# Autodesk Inventor assembly: Robot
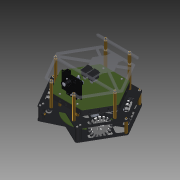
[picture p0: Inventor's stored thumbnail of the model, 180x180]
Saved by Autodesk Inventor 2015 (Build 190159000, 159)
## iProperties
Created: 2016-10-01
Part Number: Robot
Document SubType Name: Assembly
Designer: James Yelland
Author: James Yelland
## Documents named in this file (26)
- C:\Users\James Yelland\git\LJ-STAND\Design\Models\Robot\Robot.iam
- C:\Users\James Yelland\git\LJ-STAND\Design\Models\Robot\Bottom Plate.ipt
- C:\Users\James Yelland\git\LJ-STAND\Design\Models\Robot\Motor Mount.ipt
- C:\Users\James Yelland\git\LJ-STAND\Design\Models\Fasteners\Standoff 30 M-F.ipt
- C:\Users\James Yelland\git\LJ-STAND\Design\Models\Robot\LDR mount.ipt
- C:\Users\James Yelland\git\LJ-STAND\Design\Models\Robot\Laser diode mount.ipt
- C:\Users\James Yelland\git\LJ-STAND\Design\Models\Fasteners\M3x10 Screw.ipt
- C:\Users\James Yelland\git\LJ-STAND\Design\Models\Robot\Motor Support.ipt
- C:\Users\James Yelland\git\LJ-STAND\Design\Models\Fasteners\M3 Hex Nut.ipt
- C:\Users\James Yelland\git\LJ-STAND\Design\Models\Common\Imported Components\maxon_PN_0_1\maxon_PN_0_1.iam
- C:\Users\James Yelland\git\LJ-STAND\Design\Models\Fasteners\M2x4 Screw.ipt
- C:\Users\James Yelland\git\LJ-STAND\Design\Models\Robot\Light Sensor PCB.ipt
- C:\Users\James Yelland\git\LJ-STAND\Design\Models\Common\Wheel.ipt
- C:\Users\James Yelland\git\LJ-STAND\Design\Models\Robot\Middle Plate.ipt
- C:\Users\James Yelland\git\LJ-STAND\Design\Models\Fasteners\Standoff 10 M-F.ipt
- C:\Users\James Yelland\git\LJ-STAND\Design\Models\Robot\TSOP Cover Ring.ipt
- C:\Users\James Yelland\git\LJ-STAND\Design\Models\Robot\Main PCB.ipt
- C:\Users\James Yelland\git\LJ-STAND\Design\Models\Fasteners\M3x20 Screw.ipt
- C:\Users\James Yelland\git\LJ-STAND\Design\Models\Fasteners\Standoff 50 M-F.ipt
- C:\Users\James Yelland\git\LJ-STAND\Design\Models\Robot\Top Plate.ipt
- C:\Users\James Yelland\git\LJ-STAND\Design\Models\Fasteners\Standoff 20 M-F.ipt
- C:\Users\James Yelland\git\LJ-STAND\Design\Models\Robot\Handle.ipt
- C:\Users\James Yelland\git\LJ-STAND\Design\Models\Common\Laser Diode.ipt
- C:\Users\James Yelland\git\LJ-STAND\Design\Models\Common\Pixy angle bracket.ipt
- C:\Users\James Yelland\git\LJ-STAND\Design\Models\Pixy\pixy\Imported Components\Pixy(CMUcam5)\Pixy(CMUcam5).iam
- C:\Users\James Yelland\git\LJ-STAND\Design\Models\Common\Toggle switch.ipt
## Components (102 placed, 25 different names)
1. Bottom Plate:1 — Insert:1, Insert:2, Insert:3, Insert:4, Insert:5, Insert:6, Insert:7, Insert:8, Mate:1, Mate:2, Mate:3, Mate:4, Mate:5, Mate:6, Mate:7, Mate:8, Mate:9, Mate:10, Mate:11, Mate:12, Insert:9, Insert:10, Insert:11, Insert:12, Insert:31, Insert:32, Insert:33, Insert:34, Insert:35, Insert:36, Insert:37, Insert:38, Insert:39, Insert:40, Insert:45, Insert:46, Insert:47, Insert:48
2. Motor Mount:1 — Mate:2, Mate:7, Mate:8, Insert:15, Mate:13, Insert:25, Insert:26, Insert:27
3. Motor Mount:2 — Mate:1, Mate:5, Mate:6, Insert:16, Mate:14, Insert:22, Insert:23, Insert:24
4. Motor Mount:3 — Mate:3, Mate:9, Mate:10, Insert:18, Mate:15, Insert:19, Insert:20, Insert:21
5. Motor Mount:4 — Mate:4, Mate:11, Mate:12, Insert:17, Mate:16, Insert:28, Insert:29, Insert:30
6. Standoff 30 M-F:1 — Insert:3
7. Standoff 30 M-F:2 — Insert:4
8. Standoff 30 M-F:3 — Insert:2, Insert:50
9. Standoff 30 M-F:4 — Insert:1, Insert:49
10. LDR mount:1 — Insert:33, Insert:34
11. Laser diode mount:1 — Insert:31, Insert:32, Insert:93
12. M3x10 Screw:1 — Insert:5
13. M3x10 Screw:2 — Insert:7
14. M3x10 Screw:3 — Insert:6
15. M3x10 Screw:4 — Insert:8
16. Motor Support:1 — Insert:9, Insert:10, Insert:13, Insert:14
17. M3 Hex Nut:1 — Insert:13
18. M3x10 Screw:5 — Insert:12
19. M3 Hex Nut:2 — Insert:14
20. M3x10 Screw:6 — Insert:11
21. maxon_PN_0_1:1 [sub-assembly] — Insert:16, Mate:14, Mate:18, Flush:2
22. maxon_PN_0_1:2 [sub-assembly] — Insert:17, Mate:16, Mate:20, Flush:4
23. maxon_PN_0_1:3 [sub-assembly] — Insert:15, Mate:13, Mate:19, Flush:3
24. maxon_PN_0_1:4 [sub-assembly] — Insert:18, Mate:15, Mate:17, Flush:1
25. M2x4 Screw:1 — Insert:25
26. M2x4 Screw:3 — Insert:19
27. M2x4 Screw:4 — Insert:28
28. M2x4 Screw:5 — Insert:27
29. M2x4 Screw:6 — Insert:26
30. M2x4 Screw:7 — Insert:24
31. M2x4 Screw:8 — Insert:21
32. M2x4 Screw:9 — Insert:20
33. M2x4 Screw:10 — Insert:29
34. M2x4 Screw:11 — Insert:23
35. M2x4 Screw:12 — Insert:22
36. M2x4 Screw:13 — Insert:30
37. Light Sensor PCB:1 — Insert:35, Insert:36, Insert:41, Insert:42, Insert:43, Insert:44
38. M3 Hex Nut:3 — Insert:41
39. M3x10 Screw:7 — Insert:37
40. M3 Hex Nut:4 — Insert:42
41. M3x10 Screw:8 — Insert:38
42. M3 Hex Nut:5 — Insert:43
43. M3x10 Screw:9 — Insert:39
44. M3 Hex Nut:6 — Insert:44
45. M3x10 Screw:10 — Insert:40
46. M3x10 Screw:11 — Insert:45
47. M3x10 Screw:12 — Insert:46
48. M3x10 Screw:13 — Insert:47
49. M3x10 Screw:14 — Insert:48
50. Wheel:1 — Mate:18, Flush:2
51. Wheel:2 — Mate:19, Flush:3
52. Wheel:3 — Mate:17, Flush:1
53. Wheel:4 — Mate:20, Flush:4
54. Middle Plate:1 — Insert:49, Insert:50, Insert:51, Insert:52, Insert:53, Insert:54, Insert:55, Insert:56, Insert:57, Insert:58, Insert:59, Insert:60, Insert:61, Insert:62, Insert:63, Insert:64, Insert:65, Insert:66, Insert:75, Insert:76, Insert:77, Insert:78, Insert:79, Insert:80, Insert:81, Insert:82, Insert:98, Insert:99
55. M3 Hex Nut:7 — Insert:55
56. M3x10 Screw:15 — Insert:51
57. M3 Hex Nut:8 — Insert:56
58. M3x10 Screw:16 — Insert:52
59. M3 Hex Nut:9 — Insert:57
60. M3x10 Screw:17 — Insert:53
61. M3 Hex Nut:10 — Insert:58
62. M3x10 Screw:18 — Insert:54
63. Standoff 10 M-F:1 — Insert:59
64. Standoff 10 M-F:2 — Insert:60
65. Standoff 10 M-F:3 — Insert:61, Insert:67
66. Standoff 10 M-F:4 — Insert:62, Insert:68
67. M3 Hex Nut:11 — Insert:65
68. M3 Hex Nut:12 — Insert:66
69. M3 Hex Nut:13 — Insert:64
70. M3 Hex Nut:14 — Insert:63
71. TSOP Cover Ring:1 — Insert:67, Insert:68, Insert:69, Insert:70
72. Main PCB:1 — Insert:69, Insert:70, Insert:71, Insert:72, Insert:73, Insert:74, Insert:94, Insert:95
73. M3x20 Screw:1 — Insert:74
74. M3x20 Screw:2 — Insert:73
75. M3x20 Screw:3 — Insert:72
76. M3x20 Screw:4 — Insert:71
77. M3x10 Screw:19 — Insert:82
78. Standoff 50 M-F:1 — Insert:75, Insert:83
79. M3x10 Screw:20 — Insert:81
80. Standoff 50 M-F:2 — Insert:76, Insert:84
81. M3x10 Screw:21 — Insert:80
82. Standoff 50 M-F:3 — Insert:77
83. M3x10 Screw:22 — Insert:79
84. Standoff 50 M-F:4 — Insert:78
85. Top Plate:1 — Insert:83, Insert:84, Insert:85, Insert:86, Insert:91, Insert:92, Mate:21, Mate:22, Mate:23, Mate:24, Mate:25, Mate:26, Insert:100, Insert:101
86. Standoff 20 M-F:1 — Insert:85, Insert:87
87. Standoff 20 M-F:2 — Insert:86, Insert:88
88. Handle:1 — Insert:87, Insert:88, Insert:89, Insert:90
89. M3 Hex Nut:15 — Insert:89
90. M3 Hex Nut:16 — Insert:90
91. M3 Hex Nut:17 — Insert:91
92. M3 Hex Nut:18 — Insert:92
93. Laser Diode:1 — Insert:93
94. Pixy angle bracket:1 — Insert:95, Insert:96
95. Pixy angle bracket:2 — Insert:94, Insert:97
96. Pixy(CMUcam5):1 [sub-assembly] — Insert:96, Insert:97
97. Toggle switch:1 — Mate:21, Mate:25, Mate:26
98. Toggle switch:2 — Mate:22, Mate:23, Mate:24
99. Standoff 50 M-F:5 — Insert:98
100. Standoff 50 M-F:6 — Insert:99
101. M3 Hex Nut:19 — Insert:100
102. M3 Hex Nut:20 — Insert:101
## Relationships (131: Insert 101, Mate 26, Flush 4)
- Insert:1: Bottom Plate:1 ↔ Standoff 30 M-F:4
- Insert:2: Bottom Plate:1 ↔ Standoff 30 M-F:3
- Insert:3: Bottom Plate:1 ↔ Standoff 30 M-F:1
- Insert:4: Bottom Plate:1 ↔ Standoff 30 M-F:2
- Insert:5: Bottom Plate:1 ↔ M3x10 Screw:1
- Insert:6: Bottom Plate:1 ↔ M3x10 Screw:3
- Insert:7: Bottom Plate:1 ↔ M3x10 Screw:2
- Insert:8: Bottom Plate:1 ↔ M3x10 Screw:4
- Mate:1: Bottom Plate:1 ↔ Motor Mount:2
- Mate:2: Bottom Plate:1 ↔ Motor Mount:1
- Mate:3: Bottom Plate:1 ↔ Motor Mount:3
- Mate:4: Bottom Plate:1 ↔ Motor Mount:4
- Mate:5: Bottom Plate:1 ↔ Motor Mount:2
- Mate:6: Bottom Plate:1 ↔ Motor Mount:2
- Mate:7: Bottom Plate:1 ↔ Motor Mount:1
- Mate:8: Bottom Plate:1 ↔ Motor Mount:1
- Mate:9: Bottom Plate:1 ↔ Motor Mount:3
- Mate:10: Bottom Plate:1 ↔ Motor Mount:3
- Mate:11: Bottom Plate:1 ↔ Motor Mount:4
- Mate:12: Bottom Plate:1 ↔ Motor Mount:4
- Insert:9: Bottom Plate:1 ↔ Motor Support:1
- Insert:10: Bottom Plate:1 ↔ Motor Support:1
- Insert:11: Bottom Plate:1 ↔ M3x10 Screw:6
- Insert:12: Bottom Plate:1 ↔ M3x10 Screw:5
- Insert:13: Motor Support:1 ↔ M3 Hex Nut:1
- Insert:14: Motor Support:1 ↔ M3 Hex Nut:2
- Insert:15: Motor Mount:1 ↔ maxon_PN_0_1:3
- Insert:16: Motor Mount:2 ↔ maxon_PN_0_1:1
- Insert:17: Motor Mount:4 ↔ maxon_PN_0_1:2
- Insert:18: Motor Mount:3 ↔ maxon_PN_0_1:4
- Mate:13: Motor Mount:1 ↔ maxon_PN_0_1:3
- Mate:14: Motor Mount:2 ↔ maxon_PN_0_1:1
- Mate:15: Motor Mount:3 ↔ maxon_PN_0_1:4
- Mate:16: Motor Mount:4 ↔ maxon_PN_0_1:2
- Insert:19: Motor Mount:3 ↔ M2x4 Screw:3
- Insert:20: Motor Mount:3 ↔ M2x4 Screw:9
- Insert:21: Motor Mount:3 ↔ M2x4 Screw:8
- Insert:22: Motor Mount:2 ↔ M2x4 Screw:12
- Insert:23: Motor Mount:2 ↔ M2x4 Screw:11
- Insert:24: Motor Mount:2 ↔ M2x4 Screw:7
- Insert:25: Motor Mount:1 ↔ M2x4 Screw:1
- Insert:26: Motor Mount:1 ↔ M2x4 Screw:6
- Insert:27: Motor Mount:1 ↔ M2x4 Screw:5
- Insert:28: Motor Mount:4 ↔ M2x4 Screw:4
- Insert:29: Motor Mount:4 ↔ M2x4 Screw:10
- Insert:30: Motor Mount:4 ↔ M2x4 Screw:13
- Insert:31: Bottom Plate:1 ↔ Laser diode mount:1
- Insert:32: Bottom Plate:1 ↔ Laser diode mount:1
- Insert:33: Bottom Plate:1 ↔ LDR mount:1
- Insert:34: Bottom Plate:1 ↔ LDR mount:1
- Insert:35: Bottom Plate:1 ↔ Light Sensor PCB:1
- Insert:36: Bottom Plate:1 ↔ Light Sensor PCB:1
- Insert:37: Bottom Plate:1 ↔ M3x10 Screw:7
- Insert:38: Bottom Plate:1 ↔ M3x10 Screw:8
- Insert:39: Bottom Plate:1 ↔ M3x10 Screw:9
- Insert:40: Bottom Plate:1 ↔ M3x10 Screw:10
- Insert:41: Light Sensor PCB:1 ↔ M3 Hex Nut:3
- Insert:42: Light Sensor PCB:1 ↔ M3 Hex Nut:4
- Insert:43: Light Sensor PCB:1 ↔ M3 Hex Nut:5
- Insert:44: Light Sensor PCB:1 ↔ M3 Hex Nut:6
- Insert:45: Bottom Plate:1 ↔ M3x10 Screw:11
- Insert:46: Bottom Plate:1 ↔ M3x10 Screw:12
- Insert:47: Bottom Plate:1 ↔ M3x10 Screw:13
- Insert:48: Bottom Plate:1 ↔ M3x10 Screw:14
- Mate:17: maxon_PN_0_1:4 ↔ Wheel:3
- Flush:1 (-7 mm): maxon_PN_0_1:4 ↔ Wheel:3
- Mate:18: maxon_PN_0_1:1 ↔ Wheel:1
- Flush:2 (-7 mm): maxon_PN_0_1:1 ↔ Wheel:1
- Mate:19: maxon_PN_0_1:3 ↔ Wheel:2
- Flush:3 (-7 mm): maxon_PN_0_1:3 ↔ Wheel:2
- Mate:20: maxon_PN_0_1:2 ↔ Wheel:4
- Flush:4 (-7 mm): maxon_PN_0_1:2 ↔ Wheel:4
- Insert:49: Standoff 30 M-F:4 ↔ Middle Plate:1
- Insert:50: Standoff 30 M-F:3 ↔ Middle Plate:1
- Insert:51: Middle Plate:1 ↔ M3x10 Screw:15
- Insert:52: Middle Plate:1 ↔ M3x10 Screw:16
- Insert:53: Middle Plate:1 ↔ M3x10 Screw:17
- Insert:54: Middle Plate:1 ↔ M3x10 Screw:18
- Insert:55: Middle Plate:1 ↔ M3 Hex Nut:7
- Insert:56: Middle Plate:1 ↔ M3 Hex Nut:8
- Insert:57: Middle Plate:1 ↔ M3 Hex Nut:9
- Insert:58: Middle Plate:1 ↔ M3 Hex Nut:10
- Insert:59: Middle Plate:1 ↔ Standoff 10 M-F:1
- Insert:60: Middle Plate:1 ↔ Standoff 10 M-F:2
- Insert:61: Middle Plate:1 ↔ Standoff 10 M-F:3
- Insert:62: Middle Plate:1 ↔ Standoff 10 M-F:4
- Insert:63: Middle Plate:1 ↔ M3 Hex Nut:14
- Insert:64: Middle Plate:1 ↔ M3 Hex Nut:13
- Insert:65: Middle Plate:1 ↔ M3 Hex Nut:11
- Insert:66: Middle Plate:1 ↔ M3 Hex Nut:12
- Insert:67: Standoff 10 M-F:3 ↔ TSOP Cover Ring:1
- Insert:68: Standoff 10 M-F:4 ↔ TSOP Cover Ring:1
- Insert:69: TSOP Cover Ring:1 ↔ Main PCB:1
- Insert:70: TSOP Cover Ring:1 ↔ Main PCB:1
- Insert:71: Main PCB:1 ↔ M3x20 Screw:4
- Insert:72: Main PCB:1 ↔ M3x20 Screw:3
- Insert:73: Main PCB:1 ↔ M3x20 Screw:2
- Insert:74: Main PCB:1 ↔ M3x20 Screw:1
- Insert:75: Middle Plate:1 ↔ Standoff 50 M-F:1
- Insert:76: Middle Plate:1 ↔ Standoff 50 M-F:2
- Insert:77: Middle Plate:1 ↔ Standoff 50 M-F:3
- Insert:78: Middle Plate:1 ↔ Standoff 50 M-F:4
- Insert:79: Middle Plate:1 ↔ M3x10 Screw:22
- Insert:80: Middle Plate:1 ↔ M3x10 Screw:21
- Insert:81: Middle Plate:1 ↔ M3x10 Screw:20
- Insert:82: Middle Plate:1 ↔ M3x10 Screw:19
- Insert:83: Standoff 50 M-F:1 ↔ Top Plate:1
- Insert:84: Standoff 50 M-F:2 ↔ Top Plate:1
- Insert:85: Top Plate:1 ↔ Standoff 20 M-F:1
- Insert:86: Top Plate:1 ↔ Standoff 20 M-F:2
- Insert:87: Standoff 20 M-F:1 ↔ Handle:1
- Insert:88: Standoff 20 M-F:2 ↔ Handle:1
- Insert:89: Handle:1 ↔ M3 Hex Nut:15
- Insert:90: Handle:1 ↔ M3 Hex Nut:16
- Insert:91: Top Plate:1 ↔ M3 Hex Nut:17
- Insert:92: Top Plate:1 ↔ M3 Hex Nut:18
- Insert:93: Laser diode mount:1 ↔ Laser Diode:1
- Insert:94: Main PCB:1 ↔ Pixy angle bracket:2
- Insert:95: Main PCB:1 ↔ Pixy angle bracket:1
- Insert:96: Pixy angle bracket:1 ↔ Pixy(CMUcam5):1
- Insert:97: Pixy angle bracket:2 ↔ Pixy(CMUcam5):1
- Mate:21: Top Plate:1 ↔ Toggle switch:1
- Mate:22: Top Plate:1 ↔ Toggle switch:2
- Mate:23 (0.1 mm): Top Plate:1 ↔ Toggle switch:2
- Mate:24 (0.1 mm): Top Plate:1 ↔ Toggle switch:2
- Mate:25 (0.1 mm): Top Plate:1 ↔ Toggle switch:1
- Mate:26 (0.1 mm): Top Plate:1 ↔ Toggle switch:1
- Insert:98: Middle Plate:1 ↔ Standoff 50 M-F:5
- Insert:99: Middle Plate:1 ↔ Standoff 50 M-F:6
- Insert:100: Top Plate:1 ↔ M3 Hex Nut:19
- Insert:101: Top Plate:1 ↔ M3 Hex Nut:20
